# Autodesk Inventor assembly: racked
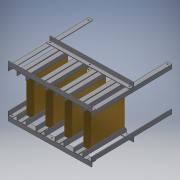
[picture p0: Inventor's stored thumbnail of the model, 180x180]
Saved by Autodesk Inventor 2017 (Build 210142000, 142)
## iProperties
Created: 2018-10-17
Part Number: racked
Document SubType Name: Assembly
Designer: ddeboer
Author: ddeboer
## Documents named in this file (4)
- C:\Users\ddeboer\Desktop\snap_holder\racked.iam
- C:\Users\ddeboer\Desktop\snap_holder\bottom.iam
- C:\Users\ddeboer\Desktop\snap_holder\snap.ipt
- C:\Users\ddeboer\Desktop\snap_holder\top.iam
## Components (6 placed, 3 different names)
1. bottom:1 [sub-assembly] — Flush:5, Flush:6, Flush:7, Mate:1, Mate:2
2. top:1 [sub-assembly] — Flush:5, Flush:6, Mate:9
3. snap:1 — Flush:7, Mate:1, Mate:2, Mate:9
4. snap:2
5. snap:3
6. snap:4
## Component patterns: (4 elements, first: snap:1)
## Relationships (6: Flush 3, Mate 3)
- Flush:5: bottom:1 ↔ top:1
- Flush:6: bottom:1 ↔ top:1
- Flush:7: bottom:1 ↔ snap:1
- Mate:1: bottom:1 ↔ snap:1
- Mate:2 (0.889 mm): bottom:1 ↔ snap:1
- Mate:9: top:1 ↔ snap:1
